# Autodesk Inventor assembly: sestava šachovnice
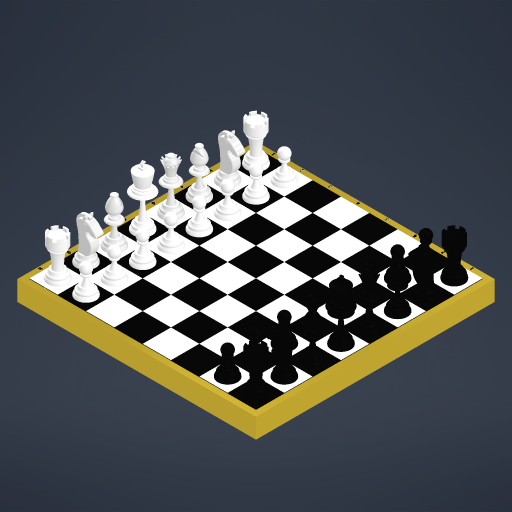
[picture p0: Inventor's stored thumbnail of the model, 512x512]
Saved by Autodesk Inventor 2023 (Build 270158000, 158)
## iProperties
Created: 2023-04-21
Part Number: sestava šachovnice
Document SubType Name: Assembly
Designer: X-DIABLO
Author: X-DIABLO
## Documents named in this file (14)
- C:\Users\X-DIABLO\OneDrive - Panská\19LCS4_Borecký Petr\2. pololetí\k odevzdání\19LBoreckyP_Závěrečná práce_Šachy\sestava šachovnice.iam
- C:\Users\X-DIABLO\OneDrive - Panská\19LCS4_Borecký Petr\2. pololetí\k odevzdání\19LBoreckyP_Závěrečná práce_Šachy\král bílý.ipt
- C:\Users\X-DIABLO\OneDrive - Panská\19LCS4_Borecký Petr\2. pololetí\k odevzdání\19LBoreckyP_Závěrečná práce_Šachy\král černý.ipt
- C:\Users\X-DIABLO\OneDrive - Panská\19LCS4_Borecký Petr\2. pololetí\k odevzdání\19LBoreckyP_Závěrečná práce_Šachy\královna bílá.ipt
- C:\Users\X-DIABLO\OneDrive - Panská\19LCS4_Borecký Petr\2. pololetí\k odevzdání\19LBoreckyP_Závěrečná práce_Šachy\královna černá.ipt
- C:\Users\X-DIABLO\OneDrive - Panská\19LCS4_Borecký Petr\2. pololetí\k odevzdání\19LBoreckyP_Závěrečná práce_Šachy\kůň bílý.ipt
- C:\Users\X-DIABLO\OneDrive - Panská\19LCS4_Borecký Petr\2. pololetí\k odevzdání\19LBoreckyP_Závěrečná práce_Šachy\kůň černý.ipt
- C:\Users\X-DIABLO\OneDrive - Panská\19LCS4_Borecký Petr\2. pololetí\k odevzdání\19LBoreckyP_Závěrečná práce_Šachy\pěšec bílý.ipt
- C:\Users\X-DIABLO\OneDrive - Panská\19LCS4_Borecký Petr\2. pololetí\k odevzdání\19LBoreckyP_Závěrečná práce_Šachy\pěšec černý.ipt
- C:\Users\X-DIABLO\OneDrive - Panská\19LCS4_Borecký Petr\2. pololetí\k odevzdání\19LBoreckyP_Závěrečná práce_Šachy\střelec bílý.ipt
- C:\Users\X-DIABLO\OneDrive - Panská\19LCS4_Borecký Petr\2. pololetí\k odevzdání\19LBoreckyP_Závěrečná práce_Šachy\střelec černý.ipt
- C:\Users\X-DIABLO\OneDrive - Panská\19LCS4_Borecký Petr\2. pololetí\k odevzdání\19LBoreckyP_Závěrečná práce_Šachy\šachovnice.ipt
- C:\Users\X-DIABLO\OneDrive - Panská\19LCS4_Borecký Petr\2. pololetí\k odevzdání\19LBoreckyP_Závěrečná práce_Šachy\věž bílá.ipt
- C:\Users\X-DIABLO\OneDrive - Panská\19LCS4_Borecký Petr\2. pololetí\k odevzdání\19LBoreckyP_Závěrečná práce_Šachy\věž černá.ipt
## Components (33 placed, 13 different names)
1. král bílý:1 — Rotational:6, Angle:5
2. král černý:1 — Rotational:14, Angle:6
3. královna bílá:1 — Rotational:5, Angle:7
4. královna černá:1 — Rotational:13, Angle:13
5. kůň bílý:1 — Rotational:3, Angle:3
6. kůň černý:1 — Rotational:1, Angle:1
7. pěšec bílý:1 — Rigid:20
8. pěšec černý:1 — Rigid:18
9. střelec bílý:1 — Rotational:4
10. střelec černý:1 — Rotational:12, Angle:14
11. šachovnice:1 — Mate:1, Mate:2, Mate:3, Rigid:17, Rigid:18, Rigid:19, Rigid:20, Rigid:21, Rigid:22, Rigid:23, Rigid:24, Rigid:25, Rigid:26, Rigid:27, Rigid:28, Rigid:29, Rigid:30, Rigid:31, Rigid:32, Rotational:1, Rotational:2, Rotational:3, Rotational:4, Rotational:5, Rotational:6, Rotational:7, Rotational:8, Rotational:9, Rotational:10, Rotational:11, Rotational:12, Rotational:13, Rotational:14, Rotational:15, Rotational:16, Angle:1, Angle:2, Angle:3, Angle:4, Angle:5, Angle:6, Angle:7, Angle:8, Angle:9, Angle:10, Angle:11, Angle:13, Angle:14, Angle:15, Angle:16
12. věž bílá:1 — Rotational:9, Angle:10
13. věž černá:1 — Rotational:10, Angle:15
14. kůň bílý:2 — Rotational:8, Angle:4
15. kůň černý:2 — Rotational:11, Angle:2
16. pěšec bílý:2 — Rigid:19
17. pěšec černý:2 — Rigid:17
18. střelec bílý:2 — Rotational:7, Angle:8
19. střelec černý:2 — Rotational:15, Angle:16
20. věž bílá:2 — Rotational:2, Angle:9
21. věž černá:2 — Rotational:16, Angle:11
22. pěšec bílý:3 — Rigid:29
23. pěšec černý:3 — Rigid:23
24. pěšec bílý:4 — Rigid:30
25. pěšec černý:4 — Rigid:21
26. pěšec bílý:5 — Rigid:27
27. pěšec černý:5 — Rigid:24
28. pěšec bílý:6 — Rigid:32
29. pěšec černý:6 — Rigid:22
30. pěšec bílý:7 — Rigid:31
31. pěšec černý:7 — Rigid:26
32. pěšec bílý:8 — Rigid:28
33. pěšec černý:8 — Rigid:25
## Relationships (50: WeldJoint 16, RevoluteJoint 16, Angle 15, Mate 3)
- Mate:1: šachovnice:1
- Mate:2: šachovnice:1
- Mate:3: šachovnice:1
- Rigid:17 [WeldJoint]: šachovnice:1 ↔ pěšec černý:2
- Rigid:18 [WeldJoint]: pěšec černý:1 ↔ šachovnice:1
- Rigid:19 [WeldJoint]: šachovnice:1 ↔ pěšec bílý:2
- Rigid:20 [WeldJoint]: pěšec bílý:1 ↔ šachovnice:1
- Rigid:21 [WeldJoint]: šachovnice:1 ↔ pěšec černý:4
- Rigid:22 [WeldJoint]: šachovnice:1 ↔ pěšec černý:6
- Rigid:23 [WeldJoint]: šachovnice:1 ↔ pěšec černý:3
- Rigid:24 [WeldJoint]: šachovnice:1 ↔ pěšec černý:5
- Rigid:25 [WeldJoint]: šachovnice:1 ↔ pěšec černý:8
- Rigid:26 [WeldJoint]: šachovnice:1 ↔ pěšec černý:7
- Rigid:27 [WeldJoint]: šachovnice:1 ↔ pěšec bílý:5
- Rigid:28 [WeldJoint]: šachovnice:1 ↔ pěšec bílý:8
- Rigid:29 [WeldJoint]: šachovnice:1 ↔ pěšec bílý:3
- Rigid:30 [WeldJoint]: šachovnice:1 ↔ pěšec bílý:4
- Rigid:31 [WeldJoint]: šachovnice:1 ↔ pěšec bílý:7
- Rigid:32 [WeldJoint]: šachovnice:1 ↔ pěšec bílý:6
- Rotational:1 [RevoluteJoint]: kůň černý:1 ↔ šachovnice:1
- Rotational:2 [RevoluteJoint]: šachovnice:1 ↔ věž bílá:2
- Rotational:3 [RevoluteJoint]: kůň bílý:1 ↔ šachovnice:1
- Rotational:4 [RevoluteJoint]: střelec bílý:1 ↔ šachovnice:1
- Rotational:5 [RevoluteJoint]: královna bílá:1 ↔ šachovnice:1
- Rotational:6 [RevoluteJoint]: král bílý:1 ↔ šachovnice:1
- Rotational:7 [RevoluteJoint]: šachovnice:1 ↔ střelec bílý:2
- Rotational:8 [RevoluteJoint]: šachovnice:1 ↔ kůň bílý:2
- Rotational:9 [RevoluteJoint]: šachovnice:1 ↔ věž bílá:1
- Rotational:10 [RevoluteJoint]: šachovnice:1 ↔ věž černá:1
- Rotational:11 [RevoluteJoint]: šachovnice:1 ↔ kůň černý:2
- Rotational:12 [RevoluteJoint]: střelec černý:1 ↔ šachovnice:1
- Rotational:13 [RevoluteJoint]: královna černá:1 ↔ šachovnice:1
- Rotational:14 [RevoluteJoint]: král černý:1 ↔ šachovnice:1
- Rotational:15 [RevoluteJoint]: šachovnice:1 ↔ střelec černý:2
- Rotational:16 [RevoluteJoint]: šachovnice:1 ↔ věž černá:2
- Angle:1 (90 deg): kůň černý:1 ↔ šachovnice:1
- Angle:2 (90 deg): šachovnice:1 ↔ kůň černý:2
- Angle:3 (90 deg): kůň bílý:1 ↔ šachovnice:1
- Angle:4 (90 deg): šachovnice:1 ↔ kůň bílý:2
- Angle:5 (0 deg): král bílý:1 ↔ šachovnice:1
- Angle:6 (0 deg): král černý:1 ↔ šachovnice:1
- Angle:7 (0 deg): královna bílá:1 ↔ šachovnice:1
- Angle:8 (0 deg): šachovnice:1 ↔ střelec bílý:2
- Angle:9 (0 deg): šachovnice:1 ↔ věž bílá:2
- Angle:10 (0 deg): šachovnice:1 ↔ věž bílá:1
- Angle:11 (0 deg): šachovnice:1 ↔ věž černá:2
- Angle:13 (0 deg): královna černá:1 ↔ šachovnice:1
- Angle:14 (0 deg): střelec černý:1 ↔ šachovnice:1
- Angle:15 (0 deg): šachovnice:1 ↔ věž černá:1
- Angle:16 (180 deg): šachovnice:1 ↔ střelec černý:2
